# Autodesk Inventor assembly: StorageAssembly.ver3-1111-2020
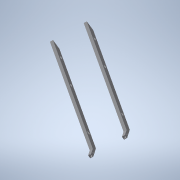
[picture p0: Inventor's stored thumbnail of the model, 180x180]
Saved by Autodesk Inventor 2021 (Build 250183000, 183)
## iProperties
Created: 2020-01-21
Part Number: StorageAssembly.ver3-1111-2020
Document SubType Name: Assembly
Designer: Power Hawks CADD
Author: Power Hawks CADD
## Documents named in this file (3)
- E:\PHRC CADD 2021\PHRC CADD\2020 Infinite Recharge\Storage\Assemblies\StorageAssembly.ver3-1111-2020.iam
- E:\PHRC CADD 2021\PHRC CADD\2020 Infinite Recharge\Shooting\Parts\AngleBrace.ver1-1111-2020.ipt
- E:\PHRC CADD 2021\PHRC CADD\2020 Infinite Recharge\Storage\Parts\BottomStorageSupport.ver1-1111-2020.ipt
## Components (4 placed, 2 different names)
1. AngleBrace.ver1-1111-2020:1
2. BottomStorageSupport.ver1-1111-2020:1
3. BottomStorageSupport.ver1-1111-2020:2
4. AngleBrace.ver1-1111-2020:2
## Relationships (4: Mate 2, Flush 2)
- [Mate]: AngleBrace.ver1-1111-2020:1 ↔ BottomStorageSupport.ver1-1111-2020:1
- [Flush]: AngleBrace.ver1-1111-2020:1 ↔ BottomStorageSupport.ver1-1111-2020:1
- [Flush]: BottomStorageSupport.ver1-1111-2020:2 ↔ AngleBrace.ver1-1111-2020:2
- [Mate]: BottomStorageSupport.ver1-1111-2020:2 ↔ AngleBrace.ver1-1111-2020:2
